# Autodesk Inventor assembly: GA12-N20微型减速直流电机3V_15RPM_8mm
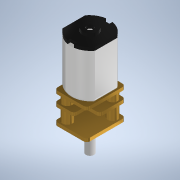
[picture p0: Inventor's stored thumbnail of the model, 180x180]
Saved by Autodesk Inventor 2022 (Build 260153000, 153)
## iProperties
Created: 2022-05-21
Part Number: GA12-N20微型减速直流电机3V_15RPM_8mm
Document SubType Name: Assembly
Designer: zhcne
Author: zhcne
## Documents named in this file (3)
- E:\Engineering_Development\SchoolProjects\2022_5_18_惯性筛_机电一体化课程设计\inertiascreen_curriculumdesign\3.Model\2.3D_Simulation\Ipt\1.偏心轮\GA12-N20微型减速直流电机3V_15RPM_8mm.iam
- E:\Engineering_Development\SchoolProjects\2022_5_18_惯性筛_机电一体化课程设计\inertiascreen_curriculumdesign\3.Model\2.3D_Simulation\Ipt\1.偏心轮\GA12-N20微型减速直流电机主机.ipt
- E:\Engineering_Development\SchoolProjects\2022_5_18_惯性筛_机电一体化课程设计\inertiascreen_curriculumdesign\3.Model\2.3D_Simulation\Ipt\1.偏心轮\GA12-N20微型减速直流电机转动轴.ipt
## Components (2 placed, 2 different names)
1. GA12-N20微型减速直流电机主机:1 — 配合:1, 配合:2
2. GA12-N20微型减速直流电机转动轴:1 — 配合:1, 配合:2
## Relationships (2: Mate 2)
- 配合:1 [Mate]: GA12-N20微型减速直流电机主机:1 ↔ GA12-N20微型减速直流电机转动轴:1
- 配合:2 [Mate]: GA12-N20微型减速直流电机主机:1 ↔ GA12-N20微型减速直流电机转动轴:1
